# Autodesk Inventor assembly: fourbarintakebearing_MIR2_MIR
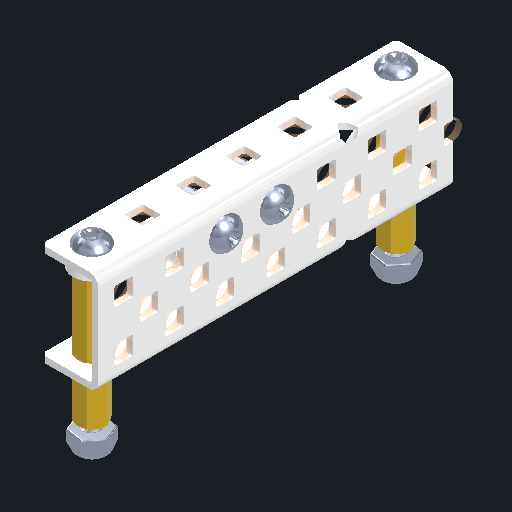
[picture p0: Inventor's stored thumbnail of the model, 512x512]
Saved by Autodesk Inventor 2023 (Build 270158000, 158)
## iProperties
Created: 2023-08-08
Part Number: fourbarintakebearing_MIR2_MIR
Document SubType Name: Assembly
Designer: srbel
Author: srbel
## Documents named in this file (12)
- C:\CAD\OverUnderCAD\Drive\fourbarintakebearing_MIR2_MIR.iam
- C:\CAD\OverUnderCAD\VEX-CAD-Inventor-1.4.0\Structure\C Channel\Aluminum 1x2x1\Alu C 1x2x1x7_MIR3_MIR.ipt
- C:\CAD\OverUnderCAD\VEX-CAD-Inventor-1.4.0\Structure\Standoff\Standoff .50.ipt
- C:\CAD\OverUnderCAD\VEX-CAD-Inventor-1.4.0\Structure\Standoff.ipt
- C:\CAD\OverUnderCAD\VEX-CAD-Inventor-1.4.0\Motion\Spacers\Spacer Nylon .313 OD\NSpacer .313 OD x .125.ipt
- C:\CAD\OverUnderCAD\VEX-CAD-Inventor-1.4.0\Motion\Spacers\Spacer Nylon .313 OD.ipt
- C:\CAD\OverUnderCAD\VEX-CAD-Inventor-1.4.0\Structure\Standoff\Standoff .75.ipt
- C:\CAD\OverUnderCAD\VEX-CAD-Inventor-1.4.0\Motion\Shaft LS\Bearing Flat_MIR5_MIR.ipt
- C:\CAD\OverUnderCAD\VEX-CAD-Inventor-1.4.0\Structure\Hardware\Screw Steel - Star\SScrew Star Threaded 1.750.ipt
- C:\CAD\OverUnderCAD\VEX-CAD-Inventor-1.4.0\Structure\Hardware\Screw Steel - Star.ipt
- C:\CAD\OverUnderCAD\VEX-CAD-Inventor-1.4.0\Structure\Hardware\Nut Thin Nylock_MIR9_MIR.ipt
- C:\CAD\OverUnderCAD\VEX-CAD-Inventor-1.4.0\Structure\Hardware\Screw Steel - Star\SScrew Star Threaded .500.ipt
## Components (16 placed, 8 different names)
1. Alu C 1x2x1x7_MIR3_MIR:1 — Insert:1, Insert:2, Insert:4, Insert:6, Insert:7, Insert:8, Insert:9, Insert:12, Insert:13, Insert:14
2. Standoff .50:1 — Insert:1, Insert:10
3. Standoff .50:2 — Insert:2, Insert:11
4. NSpacer .313 OD x .125:1 — Insert:4, Insert:3
5. Standoff .75:3 — Insert:3
6. NSpacer .313 OD x .125:2 — Insert:6, Insert:5
7. Standoff .75:4 — Insert:5
8. Bearing Flat_MIR5_MIR:1 — Insert:7, Insert:8, Insert:15, Insert:16
9. SScrew Star Threaded 1.750:1 — Insert:9
10. Nut Thin Nylock_MIR9_MIR:1 — Insert:10
11. Nut Thin Nylock_MIR9_MIR:2 — Insert:11
12. SScrew Star Threaded 1.750:2 — Insert:12
13. SScrew Star Threaded .500:3 — Insert:13
14. SScrew Star Threaded .500:4 — Insert:14
15. Nut Thin Nylock_MIR9_MIR:3 — Insert:15
16. Nut Thin Nylock_MIR9_MIR:4 — Insert:16
## Relationships (16: Insert 16)
- Insert:1: Alu C 1x2x1x7_MIR3_MIR:1 ↔ Standoff .50:1
- Insert:2: Alu C 1x2x1x7_MIR3_MIR:1 ↔ Standoff .50:2
- Insert:4: Alu C 1x2x1x7_MIR3_MIR:1 ↔ NSpacer .313 OD x .125:1
- Insert:3: NSpacer .313 OD x .125:1 ↔ Standoff .75:3
- Insert:6: Alu C 1x2x1x7_MIR3_MIR:1 ↔ NSpacer .313 OD x .125:2
- Insert:5: NSpacer .313 OD x .125:2 ↔ Standoff .75:4
- Insert:7: Alu C 1x2x1x7_MIR3_MIR:1 ↔ Bearing Flat_MIR5_MIR:1
- Insert:8: Alu C 1x2x1x7_MIR3_MIR:1 ↔ Bearing Flat_MIR5_MIR:1
- Insert:9: Alu C 1x2x1x7_MIR3_MIR:1 ↔ SScrew Star Threaded 1.750:1
- Insert:10 (1.5875 mm): Standoff .50:1 ↔ Nut Thin Nylock_MIR9_MIR:1
- Insert:11 (1.5875 mm): Standoff .50:2 ↔ Nut Thin Nylock_MIR9_MIR:2
- Insert:12: Alu C 1x2x1x7_MIR3_MIR:1 ↔ SScrew Star Threaded 1.750:2
- Insert:13: Alu C 1x2x1x7_MIR3_MIR:1 ↔ SScrew Star Threaded .500:3
- Insert:14: Alu C 1x2x1x7_MIR3_MIR:1 ↔ SScrew Star Threaded .500:4
- Insert:15: Bearing Flat_MIR5_MIR:1 ↔ Nut Thin Nylock_MIR9_MIR:3
- Insert:16: Bearing Flat_MIR5_MIR:1 ↔ Nut Thin Nylock_MIR9_MIR:4
